# Autodesk Inventor assembly: assembly
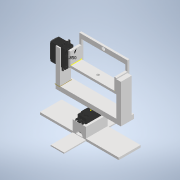
[picture p0: Inventor's stored thumbnail of the model, 180x180]
Saved by Autodesk Inventor 2021.2 (Build 252289000, 289)
## iProperties
Created: 2021-03-03
Part Number: assembly
Document SubType Name: Assembly
Designer: zayda
Author: zayda
## Documents named in this file (7)
- C:\Users\zayda\OneDrive\Desktop\general python\turret\cameraarm\v2\assembly.iam
- C:\Users\zayda\OneDrive\Desktop\general python\turret\cameraarm\v2\cameraarm.ipt
- C:\Users\zayda\OneDrive\Desktop\general python\turret\cameraarm\v2\servoarm.ipt
- C:\Users\zayda\OneDrive\Desktop\general python\turret\cameraarm\v2\servo\MG_996R.iam
- C:\Users\zayda\OneDrive\Desktop\general python\turret\cameraarm\v2\regulararm.ipt
- C:\Users\zayda\OneDrive\Desktop\general python\turret\cameraarm\v2\base.ipt
- C:\Users\zayda\OneDrive\Desktop\general python\turret\cameraarm\v2\xaxis.ipt
## Components (7 placed, 6 different names)
1. cameraarm:1 — Mate:3, Mate:4, Mate:9, Mate:10
2. servoarm:1 — Mate:1, Mate:5, Mate:7, Mate:8
3. MG_996R:1 [sub-assembly] — Mate:1, Mate:3, Mate:4, Mate:5
4. regulararm:1 — Mate:6, Mate:9, Mate:10
5. base:1 — Mate:6, Mate:7, Mate:8, Mate:14
6. xaxis:1 — Mate:11, Mate:12, Mate:13
7. MG_996R:2 [sub-assembly] — Mate:11, Mate:12, Mate:13, Mate:14
## Relationships (13: Mate 13)
- Mate:1: servoarm:1 ↔ MG_996R:1
- Mate:3: cameraarm:1 ↔ MG_996R:1
- Mate:4: cameraarm:1 ↔ MG_996R:1
- Mate:5: servoarm:1 ↔ MG_996R:1
- Mate:6: regulararm:1 ↔ base:1
- Mate:7: servoarm:1 ↔ base:1
- Mate:8: servoarm:1 ↔ base:1
- Mate:9: cameraarm:1 ↔ regulararm:1
- Mate:10: cameraarm:1 ↔ regulararm:1
- Mate:11: xaxis:1 ↔ MG_996R:2
- Mate:12: xaxis:1 ↔ MG_996R:2
- Mate:13: xaxis:1 ↔ MG_996R:2
- Mate:14: base:1 ↔ MG_996R:2
